# Autodesk Inventor assembly: all
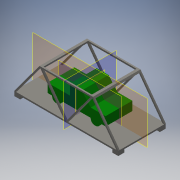
[picture p0: Inventor's stored thumbnail of the model, 180x180]
Saved by Autodesk Inventor 2019 (Build 230136000, 136)
## iProperties
Created: 2020-01-16
Part Number: all
Document SubType Name: Assembly
Designer: tguillod
Author: tguillod
## Documents named in this file (3)
- C:\Users\tguillod\Desktop\gearbox\all.iam
- C:\Users\tguillod\Desktop\gearbox\bridge.ipt
- C:\Users\tguillod\Desktop\gearbox\car.ipt
## Components (2 placed, 2 different names)
1. bridge:1 — Mate:6, Mate:7, Mate:8, Flush:1, Mate:9, Mate:10
2. car:1 — Mate:6, Mate:9, Mate:10
## Relationships (6: Mate 5, Flush 1)
- Mate:6: bridge:1 ↔ car:1
- Mate:7: bridge:1
- Mate:8: bridge:1
- Flush:1: bridge:1
- Mate:9: bridge:1 ↔ car:1
- Mate:10: bridge:1 ↔ car:1
